# Autodesk Inventor assembly: non-pivot shooter 1.1
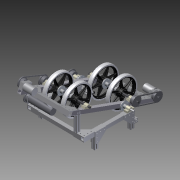
[picture p0: Inventor's stored thumbnail of the model, 180x180]
Saved by Autodesk Inventor 2011 SP1 (Build 150282100, 282)
## iProperties
Created: 2012-01-20
Part Number: non-pivot shooter 1.1
Document SubType Name: Assembly
Designer: Christopher
Author: Christopher
## Documents named in this file (22)
- C:\Users\Christopher\Documents\Christopher\FIRST\Inventor files\2012\non-pivot shooter\non-pivot shooter 1.1.iam
- C:\Users\Christopher\Documents\Christopher\FIRST\Inventor files\2012\shooter design 2\10 inch side piece.ipt
- C:\Users\Christopher\Documents\Christopher\FIRST\Inventor files\2011\Kit of Parts\Chassis\Chassis_Wheel_AndyMark_am-0420.iam
- C:\Users\Christopher\Documents\Christopher\FIRST\Inventor files\2012\shooter design 2\wheel hub.ipt
- C:\Users\Christopher\Documents\Christopher\FIRST\Inventor files\2012\shooter design 2\proxybearing.ipt
- C:\Users\Christopher\Documents\Christopher\FIRST\Inventor files\2012\shooter design 2\new vertical kicker thing.ipt
- C:\Users\Christopher\Documents\Christopher\FIRST\Inventor files\2012\shooter design 2\14 in axle.ipt
- C:\Users\Christopher\Documents\Christopher\FIRST\Inventor files\2012\shooter design 2\shooter 9 inch horizontal.ipt
- C:\Users\Christopher\Documents\Christopher\FIRST\Inventor files\2012\tower bottom second design\proxycimulator775.ipt
- C:\Users\Christopher\Documents\Christopher\FIRST\Inventor files\2012\4 wheel kicker version 1\proxy 775 motor.ipt
- C:\Users\Christopher\Documents\Christopher\FIRST\Inventor files\2012\tower bottom second design\2.5ingear proxy.ipt
- C:\Users\Christopher\Documents\Christopher\FIRST\Inventor files\2012\shooter design 2\shooterchain.ipt
- C:\Users\Christopher\Documents\Christopher\FIRST\Inventor files\2012\shooter design 2\new vertical kicker thingleft.ipt
- C:\Users\Christopher\Documents\Christopher\FIRST\Inventor files\2012\shooter design 2\12 inch middle piece.ipt
- C:\Users\Christopher\Documents\Christopher\FIRST\Inventor files\2012\shooter design 2\gearmotor proxy.ipt
- C:\Users\Christopher\Documents\Christopher\FIRST\Inventor files\2012\shooter design 2\gearmotor mounting plate.ipt
- C:\Users\Christopher\Documents\Christopher\FIRST\Inventor files\2012\shooter design 2\4.25 inch axle for shooter.ipt
- C:\Users\Christopher\Documents\Christopher\FIRST\Inventor files\2012\shooter design 2\shooter elevation change proxy chain.ipt
- C:\Users\Christopher\Documents\Christopher\FIRST\Inventor files\2012\shooter design 2\5 in shooter standoff.ipt
- C:\Users\Christopher\Documents\Christopher\FIRST\Inventor files\2012\tower first design\doorstop.ipt
- C:\Users\Christopher\Documents\Christopher\FIRST\Inventor files\2012\shooter design 2\common angle bracket.ipt
- C:\Users\Christopher\Documents\Christopher\FIRST\Inventor files\2012\shooter design 2\motor stop for turret.ipt
## Components (72 placed, 21 different names)
1. 10 inch side piece:1 — Flush:14, Flush:15, Mate:7, Mate:26, Flush:48, Flush:49, Mate:28, Flush:54, Mate:62, Mate:65, Flush:90, Flush:91, Flush:96, Insert:44, Insert:45, Insert:53, Insert:55, Insert:56, Flush:111, Insert:57
2. 10 inch side piece:2 — Mate:8, Flush:16, Flush:17, Flush:52, Flush:53, Mate:27, Mate:59, Flush:84, Flush:85, Flush:94, Insert:43, Flush:98, Mate:70, Flush:101, Insert:46, Insert:47, Insert:50, Insert:51, Insert:54
3. Chassis_Wheel_AndyMark_am-0420:1 [sub-assembly] — Insert:1
4. Chassis_Wheel_AndyMark_am-0420:2 [sub-assembly] — Insert:2
5. Chassis_Wheel_AndyMark_am-0420:3 [sub-assembly] — Insert:3
6. Chassis_Wheel_AndyMark_am-0420:4 [sub-assembly] — Insert:4
7. wheel hub:1 — Insert:1, Insert:10
8. wheel hub:2 — Insert:2, Insert:9
9. wheel hub:3 — Insert:3, Insert:11
10. wheel hub:4 — Insert:4, Insert:12
11. proxybearing:1 — Insert:8, Insert:17, Mate:25
12. proxybearing:2 — Mate:8, Flush:16, Flush:17, Insert:23, Insert:31
13. proxybearing:3 — Insert:7, Mate:24
14. proxybearing:4 — Mate:13, Flush:27, Insert:6, Insert:16, Mate:31
15. proxybearing:5 — Flush:14, Flush:15, Mate:7, Insert:30
16. proxybearing:6 — Mate:12, Flush:24, Insert:5, Flush:38, Mate:31
17. new vertical kicker thing:2 — Mate:12, Flush:24, Mate:13, Flush:27, Mate:18, Flush:36, Flush:37, Mate:20, Flush:42, Flush:43, Insert:21, Insert:24, Flush:113, Flush:114, Insert:61, Insert:63, Insert:69, Insert:74
18. 14 in axle:1 — Insert:6, Insert:7, Insert:11, Insert:12
19. 14 in axle:2 — Insert:5, Insert:8, Insert:9, Insert:10
20. shooter 9 inch horizontal:1 — Flush:38, Mate:21, Flush:113, Mate:71, Flush:114, Insert:62, Insert:64, Insert:65, Insert:75
21. shooter 9 inch horizontal:2 — Mate:18, Flush:36, Flush:37, Flush:44, Insert:67, Insert:70, Insert:72, Insert:73
22. proxycimulator775:1 — Insert:13, Mate:20, Flush:42, Flush:43, Insert:15
23. proxycimulator775:2 — Insert:14, Insert:18, Flush:45, Mate:23, Flush:46
24. proxy 775 motor:1 — Insert:13
25. proxy 775 motor:2 — Insert:14
26. 2.5ingear proxy:1 — Insert:15, Insert:19
27. 2.5ingear proxy:2 — Insert:16, Insert:28
28. 2.5ingear proxy:3 — Insert:18, Insert:20
29. 2.5ingear proxy:4 — Insert:17, Insert:27
30. shooterchain:1 — Insert:19, Insert:28
31. shooterchain:2 — Insert:20, Insert:27
32. new vertical kicker thingleft:1 — Mate:21, Flush:44, Flush:45, Mate:23, Flush:46, Mate:24, Mate:25, Insert:22, Insert:25, Insert:26, Mate:71, Insert:66, Insert:68, Insert:71, Insert:76
33. wheel hub:5 — Insert:21, Insert:24
34. wheel hub:6 — Insert:22, Insert:23, Insert:25, Insert:26
35. 12 inch middle piece:1 — Mate:26, Flush:48, Flush:49, Flush:52, Flush:53, Mate:27, Flush:55, Insert:48, Insert:49, Insert:52, Insert:58, Flush:112
36. gearmotor proxy:1 — Insert:33
37. gearmotor mounting plate:1 — Mate:28, Flush:54, Flush:55
38. 4.25 inch axle for shooter:1 — Insert:31
39. 4.25 inch axle for shooter:2 — Insert:30, Insert:32
40. 2.5ingear proxy:5 — Insert:32, Insert:35
41. 2.5ingear proxy:6 — Insert:33, Insert:34
42. shooter elevation change proxy chain:1 — Insert:34, Insert:35
43. doorstop:1 — Insert:60
44. 5 in shooter standoff:2 — Mate:59, Flush:84, Flush:85, Flush:87, Mate:60, Flush:94, Flush:109
45. 5 in shooter standoff:4 — Mate:62, Flush:100, Flush:110
46. 5 in shooter standoff:5 — Mate:65, Flush:90, Flush:91, Mate:66, Flush:92, Flush:96, Flush:99
47. 5 in shooter standoff:6 — Flush:87, Mate:60, Mate:61, Tangent:11, Tangent:12
48. 5 in shooter standoff:7 — Mate:66, Flush:92, Mate:68, Tangent:13, Tangent:14
49. doorstop:2 — Mate:68, Tangent:13, Tangent:14
50. doorstop:3 — Mate:61, Tangent:11, Tangent:12
51. common angle bracket:2 — Insert:44, Flush:99
52. common angle bracket:3 — Insert:45, Flush:100
53. common angle bracket:4 — Insert:43, Flush:98
54. common angle bracket:5 — Insert:46, Flush:102
55. 5 in shooter standoff:8 — Mate:70, Flush:101, Flush:102, Flush:108
56. common angle bracket:6 — Insert:51, Flush:108
57. common angle bracket:7 — Insert:47, Insert:48, Insert:59
58. common angle bracket:8 — Insert:54, Flush:109
59. common angle bracket:9 — Insert:49, Insert:50
60. common angle bracket:10 — Insert:52, Insert:53
61. common angle bracket:11 — Insert:56, Flush:111
62. common angle bracket:12 — Insert:57, Insert:58
63. common angle bracket:13 — Insert:55, Flush:110
64. motor stop for turret:1 — Insert:59, Flush:112, Insert:60
65. common angle bracket:14 — Insert:67, Insert:68
66. common angle bracket:15 — Insert:69, Insert:70
67. common angle bracket:16 — Insert:65, Insert:66
68. common angle bracket:17 — Insert:61, Insert:62
69. common angle bracket:18 — Insert:63, Insert:64
70. common angle bracket:19 — Insert:75, Insert:76
71. common angle bracket:20 — Insert:73, Insert:74
72. common angle bracket:21 — Insert:71, Insert:72
## Relationships (135: Insert 68, Flush 40, Mate 23, Tangent 4)
- Insert:1: Chassis_Wheel_AndyMark_am-0420:1 ↔ wheel hub:1
- Insert:2: Chassis_Wheel_AndyMark_am-0420:2 ↔ wheel hub:2
- Insert:3: Chassis_Wheel_AndyMark_am-0420:3 ↔ wheel hub:3
- Insert:4: Chassis_Wheel_AndyMark_am-0420:4 ↔ wheel hub:4
- Flush:14: 10 inch side piece:1 ↔ proxybearing:5
- Flush:15: 10 inch side piece:1 ↔ proxybearing:5
- Mate:7: 10 inch side piece:1 ↔ proxybearing:5
- Mate:8: 10 inch side piece:2 ↔ proxybearing:2
- Flush:16: 10 inch side piece:2 ↔ proxybearing:2
- Flush:17: 10 inch side piece:2 ↔ proxybearing:2
- Mate:12: proxybearing:6 ↔ new vertical kicker thing:2
- Flush:24: proxybearing:6 ↔ new vertical kicker thing:2
- Mate:13: proxybearing:4 ↔ new vertical kicker thing:2
- Flush:27: proxybearing:4 ↔ new vertical kicker thing:2
- Insert:5 (-12.7 mm): proxybearing:6 ↔ 14 in axle:2
- Insert:6 (-38.1 mm): proxybearing:4 ↔ 14 in axle:1
- Mate:18: new vertical kicker thing:2 ↔ shooter 9 inch horizontal:2
- Flush:36: new vertical kicker thing:2 ↔ shooter 9 inch horizontal:2
- Flush:37 (-63.5 mm): new vertical kicker thing:2 ↔ shooter 9 inch horizontal:2
- Flush:38 (-114.3 mm): proxybearing:6 ↔ shooter 9 inch horizontal:1
- Insert:7 (12.7 mm): proxybearing:3 ↔ 14 in axle:1
- Insert:8 (38.1 mm): proxybearing:1 ↔ 14 in axle:2
- Insert:9 (117.475 mm): wheel hub:2 ↔ 14 in axle:2
- Insert:10 (142.875 mm): wheel hub:1 ↔ 14 in axle:2
- Insert:11 (142.875 mm): wheel hub:3 ↔ 14 in axle:1
- Insert:12 (117.475 mm): wheel hub:4 ↔ 14 in axle:1
- Insert:13: proxycimulator775:1 ↔ proxy 775 motor:1
- Insert:14: proxycimulator775:2 ↔ proxy 775 motor:2
- Mate:20: new vertical kicker thing:2 ↔ proxycimulator775:1
- Flush:42: new vertical kicker thing:2 ↔ proxycimulator775:1
- Flush:43: new vertical kicker thing:2 ↔ proxycimulator775:1
- Insert:15: proxycimulator775:1 ↔ 2.5ingear proxy:1
- Insert:16: proxybearing:4 ↔ 2.5ingear proxy:2
- Insert:17: proxybearing:1 ↔ 2.5ingear proxy:4
- Insert:18: proxycimulator775:2 ↔ 2.5ingear proxy:3
- Insert:19: 2.5ingear proxy:1 ↔ shooterchain:1
- Insert:20: 2.5ingear proxy:3 ↔ shooterchain:2
- Mate:21 (63.5 mm): shooter 9 inch horizontal:1 ↔ new vertical kicker thingleft:1
- Flush:44: shooter 9 inch horizontal:2 ↔ new vertical kicker thingleft:1
- Flush:45: proxycimulator775:2 ↔ new vertical kicker thingleft:1
- Mate:23: proxycimulator775:2 ↔ new vertical kicker thingleft:1
- Flush:46: proxycimulator775:2 ↔ new vertical kicker thingleft:1
- Mate:24: proxybearing:3 ↔ new vertical kicker thingleft:1
- Mate:25: proxybearing:1 ↔ new vertical kicker thingleft:1
- Insert:21: new vertical kicker thing:2 ↔ wheel hub:5
- Insert:22: new vertical kicker thingleft:1 ↔ wheel hub:6
- Mate:26: 10 inch side piece:1 ↔ 12 inch middle piece:1
- Flush:48: 10 inch side piece:1 ↔ 12 inch middle piece:1
- Flush:49: 10 inch side piece:1 ↔ 12 inch middle piece:1
- Flush:52: 10 inch side piece:2 ↔ 12 inch middle piece:1
- Insert:23: proxybearing:2 ↔ wheel hub:6
- Flush:53: 10 inch side piece:2 ↔ 12 inch middle piece:1
- Mate:27: 10 inch side piece:2 ↔ 12 inch middle piece:1
- Insert:24: new vertical kicker thing:2 ↔ wheel hub:5
- Insert:25: new vertical kicker thingleft:1 ↔ wheel hub:6
- Insert:26: new vertical kicker thingleft:1 ↔ wheel hub:6
- Insert:27: 2.5ingear proxy:4 ↔ shooterchain:2
- Insert:28: 2.5ingear proxy:2 ↔ shooterchain:1
- Mate:28: 10 inch side piece:1 ↔ gearmotor mounting plate:1
- Flush:54: 10 inch side piece:1 ↔ gearmotor mounting plate:1
- Flush:55: 12 inch middle piece:1 ↔ gearmotor mounting plate:1
- Insert:30 (-25.4 mm): proxybearing:5 ↔ 4.25 inch axle for shooter:2
- Insert:31 (-25.4 mm): proxybearing:2 ↔ 4.25 inch axle for shooter:1
- Insert:32: 4.25 inch axle for shooter:2 ↔ 2.5ingear proxy:5
- Insert:33: gearmotor proxy:1 ↔ 2.5ingear proxy:6
- Insert:34: 2.5ingear proxy:6 ↔ shooter elevation change proxy chain:1
- Insert:35: 2.5ingear proxy:5 ↔ shooter elevation change proxy chain:1
- Mate:31 (285.75 mm): proxybearing:4 ↔ proxybearing:6
- Mate:59: 10 inch side piece:2 ↔ 5 in shooter standoff:2
- Flush:84: 10 inch side piece:2 ↔ 5 in shooter standoff:2
- Flush:85: 10 inch side piece:2 ↔ 5 in shooter standoff:2
- Flush:87: 5 in shooter standoff:2 ↔ 5 in shooter standoff:6
- Mate:60: 5 in shooter standoff:2 ↔ 5 in shooter standoff:6
- Mate:61: 5 in shooter standoff:6 ↔ doorstop:3
- Tangent:11: 5 in shooter standoff:6 ↔ doorstop:3
- Tangent:12 (22.225 mm): 5 in shooter standoff:6 ↔ doorstop:3
- Mate:62: 10 inch side piece:1 ↔ 5 in shooter standoff:4
- Mate:65: 10 inch side piece:1 ↔ 5 in shooter standoff:5
- Flush:90: 10 inch side piece:1 ↔ 5 in shooter standoff:5
- Flush:91: 10 inch side piece:1 ↔ 5 in shooter standoff:5
- Mate:66: 5 in shooter standoff:5 ↔ 5 in shooter standoff:7
- Flush:92: 5 in shooter standoff:5 ↔ 5 in shooter standoff:7
- Mate:68: 5 in shooter standoff:7 ↔ doorstop:2
- Tangent:13 (-12.7 mm): 5 in shooter standoff:7 ↔ doorstop:2
- Tangent:14 (-15.875 mm): 5 in shooter standoff:7 ↔ doorstop:2
- Flush:94: 10 inch side piece:2 ↔ 5 in shooter standoff:2
- Flush:96: 10 inch side piece:1 ↔ 5 in shooter standoff:5
- Insert:43: 10 inch side piece:2 ↔ common angle bracket:4
- Flush:98: 10 inch side piece:2 ↔ common angle bracket:4
- Insert:44: 10 inch side piece:1 ↔ common angle bracket:2
- Flush:99: 5 in shooter standoff:5 ↔ common angle bracket:2
- Insert:45: 10 inch side piece:1 ↔ common angle bracket:3
- Flush:100: 5 in shooter standoff:4 ↔ common angle bracket:3
- Mate:70: 10 inch side piece:2 ↔ 5 in shooter standoff:8
- Flush:101: 10 inch side piece:2 ↔ 5 in shooter standoff:8
- Insert:46: 10 inch side piece:2 ↔ common angle bracket:5
- Flush:102: common angle bracket:5 ↔ 5 in shooter standoff:8
- Insert:47: 10 inch side piece:2 ↔ common angle bracket:7
- Insert:48: 12 inch middle piece:1 ↔ common angle bracket:7
- Insert:49: 12 inch middle piece:1 ↔ common angle bracket:9
- Insert:50: 10 inch side piece:2 ↔ common angle bracket:9
- Insert:51: 10 inch side piece:2 ↔ common angle bracket:6
- Insert:52: 12 inch middle piece:1 ↔ common angle bracket:10
- Insert:53: 10 inch side piece:1 ↔ common angle bracket:10
- Flush:108: 5 in shooter standoff:8 ↔ common angle bracket:6
- Insert:54: 10 inch side piece:2 ↔ common angle bracket:8
- Flush:109: 5 in shooter standoff:2 ↔ common angle bracket:8
- Insert:55: 10 inch side piece:1 ↔ common angle bracket:13
- Flush:110: 5 in shooter standoff:4 ↔ common angle bracket:13
- Insert:56: 10 inch side piece:1 ↔ common angle bracket:11
- Flush:111: 10 inch side piece:1 ↔ common angle bracket:11
- Insert:57: 10 inch side piece:1 ↔ common angle bracket:12
- Insert:58: 12 inch middle piece:1 ↔ common angle bracket:12
- Insert:59: common angle bracket:7 ↔ motor stop for turret:1
- Flush:112: 12 inch middle piece:1 ↔ motor stop for turret:1
- Insert:60: doorstop:1 ↔ motor stop for turret:1
- Flush:113: new vertical kicker thing:2 ↔ shooter 9 inch horizontal:1
- Mate:71: shooter 9 inch horizontal:1 ↔ new vertical kicker thingleft:1
- Flush:114: new vertical kicker thing:2 ↔ shooter 9 inch horizontal:1
- Insert:61: new vertical kicker thing:2 ↔ common angle bracket:17
- Insert:62: shooter 9 inch horizontal:1 ↔ common angle bracket:17
- Insert:63: new vertical kicker thing:2 ↔ common angle bracket:18
- Insert:64: shooter 9 inch horizontal:1 ↔ common angle bracket:18
- Insert:65: shooter 9 inch horizontal:1 ↔ common angle bracket:16
- Insert:66: new vertical kicker thingleft:1 ↔ common angle bracket:16
- Insert:67: shooter 9 inch horizontal:2 ↔ common angle bracket:14
- Insert:68: new vertical kicker thingleft:1 ↔ common angle bracket:14
- Insert:69: new vertical kicker thing:2 ↔ common angle bracket:15
- Insert:70: shooter 9 inch horizontal:2 ↔ common angle bracket:15
- Insert:71: new vertical kicker thingleft:1 ↔ common angle bracket:21
- Insert:72: shooter 9 inch horizontal:2 ↔ common angle bracket:21
- Insert:73: shooter 9 inch horizontal:2 ↔ common angle bracket:20
- Insert:74: new vertical kicker thing:2 ↔ common angle bracket:20
- Insert:75: shooter 9 inch horizontal:1 ↔ common angle bracket:19
- Insert:76: new vertical kicker thingleft:1 ↔ common angle bracket:19
